# Autodesk Inventor assembly: Toyota Yaris USB Assembly
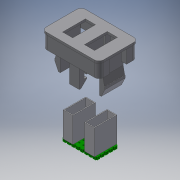
[picture p0: Inventor's stored thumbnail of the model, 180x180]
Saved by Autodesk Inventor 2018.1 (Build 221171000, 171)
## iProperties
Created: 2017-10-18
Part Number: Toyota Yaris USB Assembly
Document SubType Name: Assembly
Designer: xdlea
Author: xdlea
## Documents named in this file (4)
- D:\Users\Andrew\OneDrive\3D Models\Toyota Yaris Aux Cap\Toyota Yaris USB Assembly.iam
- D:\Users\Andrew\OneDrive\3D Models\Toyota Yaris Aux Cap\Toyota Yaris USB Cover.ipt
- D:\Users\Andrew\OneDrive\3D Models\Toyota Yaris Aux Cap\Toyota Yaris USB PCB.ipt
- D:\Users\Andrew\OneDrive\3D Models\Toyota Yaris Aux Cap\Female USB SMT.ipt
## Components (4 placed, 3 different names)
1. Toyota Yaris USB Cover:1 — Mate:1, Mate:2, Flush:1
2. Toyota Yaris USB PCB:1 — Mate:3, Mate:4, Mate:5, Mate:6, Mate:7
3. Female USB SMT:1 — Flush:2, Flush:3, Mate:6
4. Female USB SMT:2 — Flush:2, Flush:3, Mate:5, Mate:7
## Relationships (10: Mate 7, Flush 3)
- Mate:1: Toyota Yaris USB Cover:1
- Mate:2: Toyota Yaris USB Cover:1
- Flush:1: Toyota Yaris USB Cover:1
- Mate:3: Toyota Yaris USB PCB:1
- Mate:4: Toyota Yaris USB PCB:1
- Flush:2: Female USB SMT:1 ↔ Female USB SMT:2
- Flush:3: Female USB SMT:1 ↔ Female USB SMT:2
- Mate:5: Toyota Yaris USB PCB:1 ↔ Female USB SMT:2
- Mate:6: Toyota Yaris USB PCB:1 ↔ Female USB SMT:1
- Mate:7: Toyota Yaris USB PCB:1 ↔ Female USB SMT:2
